# Autodesk Inventor assembly: Differential_bord
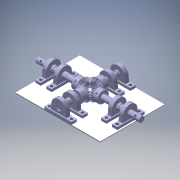
[picture p0: Inventor's stored thumbnail of the model, 180x180]
Saved by Autodesk Inventor 2018.1 (Build 221171000, 171)
## iProperties
Created: 2017-09-21
Part Number: Differential_bord
Material: 一般
Document SubType Name: Assembly
Designer: Kakeru Yamashita
Author: Kakeru Yamashita
## Documents named in this file (6)
- C:\Users\Kakeru Yamashita\Desktop\fr03\Differential_bord.iam
- C:\Users\Kakeru Yamashita\Desktop\fr03\base_diff_02.ipt
- C:\Users\Kakeru Yamashita\Desktop\fr03\Differential_Gear_Box.iam
- C:\Users\Kakeru Yamashita\Desktop\fr03\support_bearing.ipt
- C:\Users\Kakeru Yamashita\Desktop\fr03\Shaft_satellite 2.ipt
- C:\Users\Kakeru Yamashita\Desktop\fr03\differential_shaft.ipt
## Components (14 placed, 5 different names)
1. base_diff_02:1 — メイト:1, メイト:2, メイト:3, メイト:4, メイト:5, メイト:6, メイト:7, メイト:8, メイト:9, メイト:10, メイト:11, メイト:12, メイト:13, メイト:14, メイト:15, メイト:16, メイト:17, メイト:18, メイト:19, メイト:20, メイト:21, メイト:22, メイト:23, メイト:24, メイト:27, フラッシュ:1
2. Differential_Gear_Box:1 [sub-assembly] — メイト:28, メイト:29, メイト:31, メイト:33, メイト:34, メイト:35
3. support_bearing:1 — メイト:1, メイト:2, メイト:13
4. support_bearing:2 — メイト:3, メイト:4, メイト:14, メイト:30
5. support_bearing:3 — メイト:11, メイト:12, メイト:15, メイト:26
6. support_bearing:4 — メイト:9, メイト:10, メイト:16
7. support_bearing:5 — メイト:5, メイト:6, メイト:18, メイト:32
8. support_bearing:6 — メイト:21, メイト:22, メイト:23
9. support_bearing:7 — メイト:7, メイト:8, メイト:17
10. support_bearing:8 — メイト:19, メイト:20, メイト:24, メイト:25
11. Shaft_satellite 2:1 — メイト:25, メイト:28, メイト:35
12. Shaft_satellite 2:2 — メイト:26, メイト:34
13. differential_shaft:1 — メイト:29, メイト:30, メイト:31
14. differential_shaft:2 — メイト:32, メイト:33
## Relationships (36: Mate 35, Flush 1)
- メイト:1 [Mate]: base_diff_02:1 ↔ support_bearing:1
- メイト:2 [Mate]: base_diff_02:1 ↔ support_bearing:1
- メイト:3 [Mate]: base_diff_02:1 ↔ support_bearing:2
- メイト:4 [Mate]: base_diff_02:1 ↔ support_bearing:2
- メイト:5 [Mate]: base_diff_02:1 ↔ support_bearing:5
- メイト:6 [Mate]: base_diff_02:1 ↔ support_bearing:5
- メイト:7 [Mate]: base_diff_02:1 ↔ support_bearing:7
- メイト:8 [Mate]: base_diff_02:1 ↔ support_bearing:7
- メイト:9 [Mate]: base_diff_02:1 ↔ support_bearing:4
- メイト:10 [Mate]: base_diff_02:1 ↔ support_bearing:4
- メイト:11 [Mate]: base_diff_02:1 ↔ support_bearing:3
- メイト:12 [Mate]: base_diff_02:1 ↔ support_bearing:3
- メイト:13 [Mate]: base_diff_02:1 ↔ support_bearing:1
- メイト:14 [Mate]: base_diff_02:1 ↔ support_bearing:2
- メイト:15 [Mate]: base_diff_02:1 ↔ support_bearing:3
- メイト:16 [Mate]: base_diff_02:1 ↔ support_bearing:4
- メイト:17 [Mate]: base_diff_02:1 ↔ support_bearing:7
- メイト:18 [Mate]: base_diff_02:1 ↔ support_bearing:5
- メイト:19 [Mate]: base_diff_02:1 ↔ support_bearing:8
- メイト:20 [Mate]: base_diff_02:1 ↔ support_bearing:8
- メイト:21 [Mate]: base_diff_02:1 ↔ support_bearing:6
- メイト:22 [Mate]: base_diff_02:1 ↔ support_bearing:6
- メイト:23 [Mate]: base_diff_02:1 ↔ support_bearing:6
- メイト:24 [Mate]: base_diff_02:1 ↔ support_bearing:8
- メイト:25 [Mate]: support_bearing:8 ↔ Shaft_satellite 2:1
- メイト:26 [Mate]: support_bearing:3 ↔ Shaft_satellite 2:2
- メイト:27 [Mate]: base_diff_02:1
- フラッシュ:1 [Flush]: base_diff_02:1
- メイト:28 [Mate]: Differential_Gear_Box:1 ↔ Shaft_satellite 2:1
- メイト:29 [Mate]: Differential_Gear_Box:1 ↔ differential_shaft:1
- メイト:30 [Mate]: support_bearing:2 ↔ differential_shaft:1
- メイト:31 [Mate]: Differential_Gear_Box:1 ↔ differential_shaft:1
- メイト:32 [Mate]: support_bearing:5 ↔ differential_shaft:2
- メイト:33 [Mate]: Differential_Gear_Box:1 ↔ differential_shaft:2
- メイト:34 [Mate]: Differential_Gear_Box:1 ↔ Shaft_satellite 2:2
- メイト:35 [Mate]: Differential_Gear_Box:1 ↔ Shaft_satellite 2:1
